# Autodesk Inventor assembly: Combustion Chamber Assembly
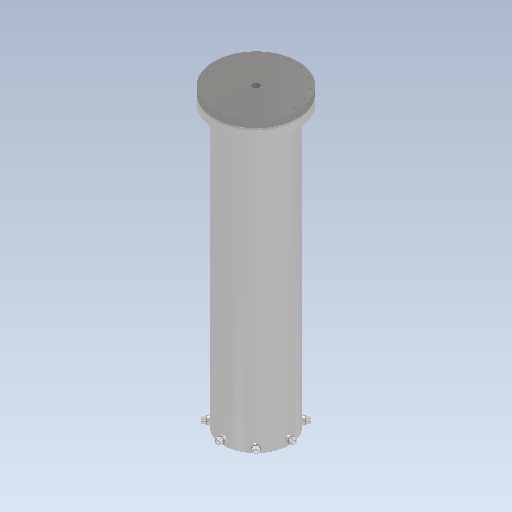
[picture p0: Inventor's stored thumbnail of the model, 512x512]
Saved by Autodesk Inventor 2021 (Build 250183000, 183)
## iProperties
Created: 2021-02-14
Part Number: Combustion Chamber Assembly
Document SubType Name: Assembly
Designer: alexc
Mass: 14919.3 g
Surface Area: 11748.8 cm^2
Volume: 9084.34 cm^3
Density: 1.64231 g/cm^3
Author: alexc
## Documents named in this file (9)
- C:\Users\alexc\OneDrive\Desktop\ATLAS\ODSY-0003 (COMBUSTION CHAMBER)\ODSY-0003.iam
- C:\Users\alexc\OneDrive\Desktop\ATLAS\ODSY-0003 (COMBUSTION CHAMBER)\ODSY-0003-400 (CC HOUSING)\Combustion Chamber.ipt
- C:\Users\alexc\OneDrive\Desktop\ATLAS\ODSY-0003 (COMBUSTION CHAMBER)\ODSY-0003-400 (CC HOUSING)\Injector Plate Retainer Ring.ipt
- C:\Users\alexc\OneDrive\Desktop\ATLAS\ODSY-0003 (COMBUSTION CHAMBER)\ODSY-0003-300 (FUEL GRAIN)\Fuel Grain.iam
- C:\Users\alexc\OneDrive\Desktop\ATLAS\ODSY-0003 (COMBUSTION CHAMBER)\ODSY-0003-200 (INJECTOR)\ODSY-0003-200.iam
- C:\Users\alexc\OneDrive\Desktop\ATLAS\ODSY-0003 (COMBUSTION CHAMBER)\ODSY-0003-200 (INJECTOR)\90945A760.ipt
- C:\Users\alexc\OneDrive\Desktop\ATLAS\ODSY-0003 (COMBUSTION CHAMBER)\Spacers.ipt
- C:\Users\alexc\OneDrive\Desktop\ATLAS\ODSY-0003 (COMBUSTION CHAMBER)\92196A540.ipt
- C:\Users\alexc\OneDrive\Desktop\ATLAS\ODSY-0003 (COMBUSTION CHAMBER)\ODSY-0003-100 (NOZZLE)\ODSY-0003-100.iam
## Components (29 placed, 8 different names)
1. Injector Plate Retainer Ring:1 — Mate:12, Flush:2, Mate:33, Mate:41
2. Fuel Grain:1 [sub-assembly] — Mate:26, Flush:1, Mate:40, Mate:82
3. ODSY-0003-200:1 [sub-assembly] — Mate:38, Mate:40, Mate:41
4. Combustion Chamber:1 — Mate:8, Mate:9, Mate:12, Angle:1, Mate:26, Flush:2, Mate:33, Mate:38, Mate:69, Mate:70, Mate:80, Mate:81
5. ODSY-0003-100:1 [sub-assembly] — Mate:80, Mate:81, Mate:82
6. Spacers:1 — Mate:69, Mate:70, Mate:71, Mate:72
7. Spacers:2
8. Spacers:3
9. Spacers:4
10. Spacers:5
11. Spacers:6
12. Spacers:7
13. Spacers:8
14. 92196A540:1 — Mate:73, Mate:74, Angle:4
15. 92196A540:2
16. 92196A540:3
17. 92196A540:4
18. 92196A540:5
19. 92196A540:6
20. 92196A540:7
21. 92196A540:8
22. 90945A760:54 — Mate:71, Mate:72, Mate:73, Mate:74
23. 90945A760:55
24. 90945A760:56
25. 90945A760:57
26. 90945A760:58
27. 90945A760:59
28. 90945A760:60
29. 90945A760:61
## Component patterns: (8 elements, first: Spacers:1), (8 elements, first: 92196A540:1), (8 elements, first: 90945A760:54)
## Relationships (21: Mate 17, Angle 2, Flush 2)
- Mate:8: Combustion Chamber:1
- Mate:9: Combustion Chamber:1
- Mate:12: Injector Plate Retainer Ring:1 ↔ Combustion Chamber:1
- Angle:1 (0 deg): Combustion Chamber:1
- Mate:26: Fuel Grain:1 ↔ Combustion Chamber:1
- Flush:1: Fuel Grain:1
- Flush:2: Injector Plate Retainer Ring:1 ↔ Combustion Chamber:1
- Mate:33: Injector Plate Retainer Ring:1 ↔ Combustion Chamber:1
- Mate:38: ODSY-0003-200:1 ↔ Combustion Chamber:1
- Mate:40: Fuel Grain:1 ↔ ODSY-0003-200:1
- Mate:41: Injector Plate Retainer Ring:1 ↔ ODSY-0003-200:1
- Mate:69: Combustion Chamber:1 ↔ Spacers:1
- Mate:70: Combustion Chamber:1 ↔ Spacers:1
- Mate:71: Spacers:1 ↔ 90945A760:54
- Mate:72: Spacers:1 ↔ 90945A760:54
- Mate:73: 92196A540:1 ↔ 90945A760:54
- Mate:74: 92196A540:1 ↔ 90945A760:54
- Angle:4 (0 deg): 92196A540:1
- Mate:80: Combustion Chamber:1 ↔ ODSY-0003-100:1
- Mate:81: Combustion Chamber:1 ↔ ODSY-0003-100:1
- Mate:82: Fuel Grain:1 ↔ ODSY-0003-100:1
